# Autodesk Inventor assembly: am_test1
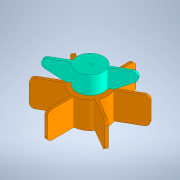
[picture p0: Inventor's stored thumbnail of the model, 180x180]
Saved by Autodesk Inventor 2021 (Build 250183000, 183)
## iProperties
Created: 2023-05-04
Part Number: am_test1
Document SubType Name: Assembly
Designer: assman
Author: assman
## Documents named in this file (3)
- C:\dev\3Dmodels\catfeeder\am_test1.iam
- C:\dev\3Dmodels\catfeeder\sketch_for_propeller.ipt
- C:\dev\3Dmodels\catfeeder\top_propeller.ipt
## Components (2 placed, 2 different names)
1. sketch_for_propeller:1 — Rotational:1
2. top_propeller:1 — Rotational:1
## Relationships (1: RevoluteJoint 1)
- Rotational:1 [RevoluteJoint] (-1 mm): sketch_for_propeller:1 ↔ top_propeller:1
